# Autodesk Inventor assembly: Main Assembily
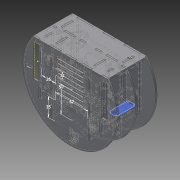
[picture p0: Inventor's stored thumbnail of the model, 180x180]
Saved by Autodesk Inventor 2015 (Build 190159000, 159)
## iProperties
Created: 2014-11-10
Part Number: Main Assembily
Document SubType Name: Assembly
Designer: karl
Author: karl
## Documents named in this file (17)
- C:\Users\karl\Documents\GitHub\Workshop_Robots\Mechanical\Rev.1\Main Assembily.iam
- C:\Users\karl\Documents\GitHub\Workshop_Robots\Mechanical\Rev.1\Base Plate.ipt
- C:\Users\karl\Documents\GitHub\Workshop_Robots\Mechanical\Rev.1\Motor support.ipt
- C:\Users\karl\Documents\GitHub\Workshop_Robots\Mechanical\Rev.1\Motor support plate.ipt
- C:\Users\karl\Documents\GitHub\Workshop_Robots\Mechanical\Rev.1\Lower bottom.ipt
- C:\Users\karl\Documents\GitHub\Workshop_Robots\Mechanical\Rev.1\Bottom battery holder.ipt
- C:\Users\karl\Documents\GitHub\Workshop_Robots\Mechanical\Standered Parts\Micro Gear motor.ipt
- C:\Users\karl\Documents\GitHub\Workshop_Robots\Mechanical\Standered Parts\Mid Plate.ipt
- C:\Users\karl\Documents\GitHub\Workshop_Robots\Mechanical\Rev.1\Battery holder.ipt
- C:\Users\karl\Documents\GitHub\Workshop_Robots\Mechanical\Rev.1\Board holders.ipt
- C:\Users\karl\Documents\GitHub\Workshop_Robots\Mechanical\Rev.1\Battey latch.ipt
- C:\Users\karl\Documents\GitHub\Workshop_Robots\Mechanical\Rev.1\Bolt Cradel.ipt
- C:\Users\karl\Documents\GitHub\Workshop_Robots\Mechanical\Rev.1\Cradel holder.ipt
- C:\Users\karl\Documents\GitHub\Workshop_Robots\Mechanical\Rev.1\Top Plate.ipt
- C:\Users\karl\Documents\GitHub\Workshop_Robots\Mechanical\Rev.1\Out side rib.ipt
- C:\Users\karl\Documents\GitHub\Workshop_Robots\Mechanical\Rev.1\Mid rib support.ipt
- C:\Users\karl\Documents\GitHub\Workshop_Robots\Mechanical\Rev.1\Frount.ipt
## Components (25 placed, 16 different names)
1. Base Plate:1 — Flush:1, Flush:2, Flush:3, Flush:4, Mate:1, Flush:5, Mate:2, Mate:4, Mate:5, Mate:6, Mate:7, Flush:9, Mate:8, Mate:9, Mate:10, Flush:12, Mate:16, Mate:36, Flush:23, Mate:39, Mate:41, Mate:44
2. Motor support:1 — Flush:1, Flush:2, Flush:3, Flush:10, Mate:12, Mate:13, Flush:17, Flush:18, Flush:22, Mate:35
3. Motor support plate:1 — Flush:4, Mate:1, Flush:5, Flush:6, Flush:7, Flush:8, Mate:11, Mate:14
4. Lower bottom:1 — Mate:2, Flush:6, Mate:11
5. Bottom battery holder:1 — Mate:4, Mate:5, Mate:6, Flush:11, Mate:17
6. Motor support plate:2 — Flush:7, Flush:8, Mate:7, Mate:15
7. Motor support:2 — Flush:9, Flush:10, Mate:8, Flush:13, Mate:20, Mate:21, Flush:14, Mate:31, Mate:32, Mate:33, Mate:37, Mate:38
8. Bottom battery holder:2 — Mate:9, Mate:10, Flush:11, Mate:18
9. Micro Gear motor:1 — Mate:12, Mate:13, Mate:14
10. Mid Plate:1 — Mate:15, Flush:12, Mate:16, Mate:19, Mate:22, Mate:23, Mate:24, Mate:25, Mate:26, Mate:27, Mate:28, Mate:40, Mate:43, Mate:45, Flush:25
11. Battery holder:1 — Mate:17, Mate:18
12. Board holders:1 — Mate:19, Flush:13, Mate:20, Mate:30
13. Board holders:2 — Mate:21, Mate:22, Flush:14
14. Battey latch:1 — Mate:23, Mate:24, Mate:25, Flush:15, Flush:16
15. Battey latch:2 — Mate:26, Flush:15, Flush:16
16. Board holders:3 — Mate:27, Flush:17, Flush:18, Flush:19, Flush:20, Mate:29
17. Board holders:4 — Flush:19, Flush:20, Mate:28
18. Bolt Cradel:1 — Mate:29, Mate:30, Mate:34
19. Cradel holder:1 — Mate:31, Mate:32, Mate:33, Mate:34, Flush:21
20. Cradel holder:2 — Flush:21, Flush:22, Mate:35
21. Top Plate:1 — Mate:36, Mate:37, Flush:23
22. Out side rib:1 — Mate:38, Mate:39, Mate:40, Flush:24, Mate:42
23. Mid rib support:1 — Mate:41, Flush:24, Mate:42
24. Out side rib:2 — Mate:43, Mate:44, Mate:45
25. Frount:1 — Flush:25
## Relationships (69: Mate 44, Flush 25)
- Flush:1: Base Plate:1 ↔ Motor support:1
- Flush:2: Base Plate:1 ↔ Motor support:1
- Flush:3: Base Plate:1 ↔ Motor support:1
- Flush:4: Base Plate:1 ↔ Motor support plate:1
- Mate:1: Base Plate:1 ↔ Motor support plate:1
- Flush:5: Base Plate:1 ↔ Motor support plate:1
- Mate:2: Base Plate:1 ↔ Lower bottom:1
- Flush:6: Motor support plate:1 ↔ Lower bottom:1
- Mate:4: Base Plate:1 ↔ Bottom battery holder:1
- Mate:5: Base Plate:1 ↔ Bottom battery holder:1
- Mate:6: Base Plate:1 ↔ Bottom battery holder:1
- Flush:7: Motor support plate:1 ↔ Motor support plate:2
- Flush:8: Motor support plate:1 ↔ Motor support plate:2
- Mate:7: Base Plate:1 ↔ Motor support plate:2
- Flush:9: Base Plate:1 ↔ Motor support:2
- Flush:10: Motor support:1 ↔ Motor support:2
- Mate:8: Base Plate:1 ↔ Motor support:2
- Mate:9: Base Plate:1 ↔ Bottom battery holder:2
- Mate:10: Base Plate:1 ↔ Bottom battery holder:2
- Flush:11: Bottom battery holder:1 ↔ Bottom battery holder:2
- Mate:11: Motor support plate:1 ↔ Lower bottom:1
- Mate:12: Motor support:1 ↔ Micro Gear motor:1
- Mate:13: Motor support:1 ↔ Micro Gear motor:1
- Mate:14: Motor support plate:1 ↔ Micro Gear motor:1
- Mate:15: Motor support plate:2 ↔ Mid Plate:1
- Flush:12: Base Plate:1 ↔ Mid Plate:1
- Mate:16: Base Plate:1 ↔ Mid Plate:1
- Mate:17: Bottom battery holder:1 ↔ Battery holder:1
- Mate:18: Bottom battery holder:2 ↔ Battery holder:1
- Mate:19: Mid Plate:1 ↔ Board holders:1
- Flush:13: Motor support:2 ↔ Board holders:1
- Mate:20: Motor support:2 ↔ Board holders:1
- Mate:21: Motor support:2 ↔ Board holders:2
- Mate:22: Mid Plate:1 ↔ Board holders:2
- Flush:14: Motor support:2 ↔ Board holders:2
- Mate:23: Mid Plate:1 ↔ Battey latch:1
- Mate:24: Mid Plate:1 ↔ Battey latch:1
- Mate:25: Mid Plate:1 ↔ Battey latch:1
- Mate:26: Mid Plate:1 ↔ Battey latch:2
- Flush:15: Battey latch:1 ↔ Battey latch:2
- Flush:16: Battey latch:1 ↔ Battey latch:2
- Mate:27: Mid Plate:1 ↔ Board holders:3
- Flush:17: Motor support:1 ↔ Board holders:3
- Flush:18: Motor support:1 ↔ Board holders:3
- Flush:19: Board holders:3 ↔ Board holders:4
- Flush:20: Board holders:3 ↔ Board holders:4
- Mate:28: Mid Plate:1 ↔ Board holders:4
- Mate:29: Board holders:3 ↔ Bolt Cradel:1
- Mate:30: Board holders:1 ↔ Bolt Cradel:1
- Mate:31: Motor support:2 ↔ Cradel holder:1
- Mate:32: Motor support:2 ↔ Cradel holder:1
- Mate:33: Motor support:2 ↔ Cradel holder:1
- Mate:34: Bolt Cradel:1 ↔ Cradel holder:1
- Flush:21: Cradel holder:1 ↔ Cradel holder:2
- Flush:22: Motor support:1 ↔ Cradel holder:2
- Mate:35: Motor support:1 ↔ Cradel holder:2
- Mate:36: Base Plate:1 ↔ Top Plate:1
- Mate:37: Motor support:2 ↔ Top Plate:1
- Flush:23: Base Plate:1 ↔ Top Plate:1
- Mate:38: Motor support:2 ↔ Out side rib:1
- Mate:39: Base Plate:1 ↔ Out side rib:1
- Mate:40: Mid Plate:1 ↔ Out side rib:1
- Mate:41: Base Plate:1 ↔ Mid rib support:1
- Flush:24: Out side rib:1 ↔ Mid rib support:1
- Mate:42: Out side rib:1 ↔ Mid rib support:1
- Mate:43: Mid Plate:1 ↔ Out side rib:2
- Mate:44: Base Plate:1 ↔ Out side rib:2
- Mate:45: Mid Plate:1 ↔ Out side rib:2
- Flush:25: Mid Plate:1 ↔ Frount:1
